# Autodesk Inventor assembly: Knee_LeftRear_MIR
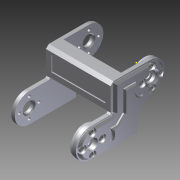
[picture p0: Inventor's stored thumbnail of the model, 180x180]
Saved by Autodesk Inventor 2015 (Build 190159000, 159)
## iProperties
Created: 2015-05-22
Part Number: Knee_LeftRear_MIR
Document SubType Name: Assembly
Designer: Quinn
Author: Quinn
## Documents named in this file (4)
- C:\Users\Quinn\Desktop\3DCNC Design\InventorModels\Assemblies\Knee_LeftRear_MIR.iam
- C:\Users\Quinn\Desktop\3DCNC Design\InventorModels\Electronics\Servo\ServoHornPlastic_MIR.ipt
- C:\Users\Quinn\Desktop\3DCNC Design\InventorModels\Plastics\KneeUpgradeMk3.1Blank_MIR.ipt
- C:\Users\Quinn\Desktop\3DCNC Design\InventorModels\Assemblies\Knee_RightFront\Design Accelerator\Bolted Connection2_MIR.iam
## Components (4 placed, 3 different names)
1. ServoHornPlastic_MIR:1 — Insert:1
2. ServoHornPlastic_MIR:2 — Mate:4, Mate:3, Insert:2
3. KneeUpgradeMk3.1Blank_MIR:1 — Mate:4, Mate:3, Insert:2, Insert:1, Mate:6, Mate:5
4. Bolted Connection2_MIR:1 [sub-assembly] — Mate:6, Mate:5
## Relationships (6: Mate 3, Insert 2, Flush 1)
- Mate:4: ServoHornPlastic_MIR:2 ↔ KneeUpgradeMk3.1Blank_MIR:1
- Mate:3: ServoHornPlastic_MIR:2 ↔ KneeUpgradeMk3.1Blank_MIR:1
- Insert:2: ServoHornPlastic_MIR:2 ↔ KneeUpgradeMk3.1Blank_MIR:1
- Insert:1: ServoHornPlastic_MIR:1 ↔ KneeUpgradeMk3.1Blank_MIR:1
- Mate:6: KneeUpgradeMk3.1Blank_MIR:1 ↔ Bolted Connection2_MIR:1
- Mate:5 [Flush]: KneeUpgradeMk3.1Blank_MIR:1 ↔ Bolted Connection2_MIR:1
